# Autodesk Inventor assembly: Part_Truot_T_Nhom
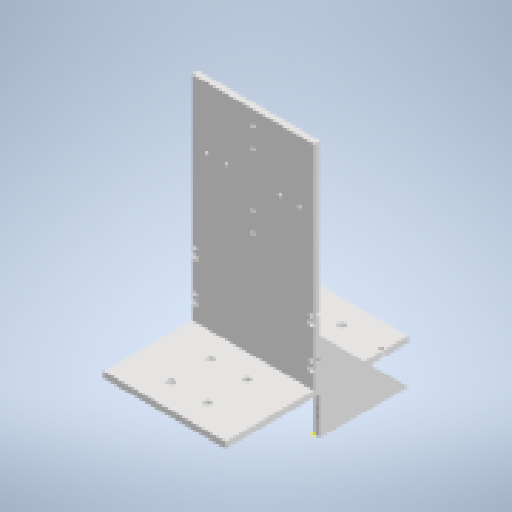
[picture p0: Inventor's stored thumbnail of the model, 512x512]
Saved by Autodesk Inventor 2023 (Build 270158000, 158)
## iProperties
Created: 2025-04-17
Part Number: Part_Truot_T_Nhom
Document SubType Name: Assembly
Designer: huyqu
Author: huyqu
## Documents named in this file (4)
- E:\TAI LIEU\Final_Project\DONE\CoCauTrucZ\Part_Truot_T_Nhom.iam
- E:\TAI LIEU\Final_Project\DONE\CoCauTrucZ\350x200(10li).ipt
- E:\TAI LIEU\Final_Project\DONE\CoCauTrucZ\145x145(li).ipt
- E:\TAI LIEU\Final_Project\DONE\CoCauTrucZ\200x300(10li).ipt
## Components (4 placed, 3 different names)
1. 145x145(li):1 — Mate:1, Mate:2
2. 145x145(li):2 — Mate:3, Mate:4
3. 200x300(10li):1 — Mate:5, Mate:6
4. 350x200(10li):1 — Mate:1, Mate:2, Mate:3, Mate:4, Mate:5, Mate:6
## Relationships (6: Mate 6)
- Mate:1: 145x145(li):1 ↔ 350x200(10li):1
- Mate:2: 145x145(li):1 ↔ 350x200(10li):1
- Mate:3: 145x145(li):2 ↔ 350x200(10li):1
- Mate:4: 145x145(li):2 ↔ 350x200(10li):1
- Mate:5: 200x300(10li):1 ↔ 350x200(10li):1
- Mate:6: 200x300(10li):1 ↔ 350x200(10li):1
